# Autodesk Inventor assembly: bladesupport
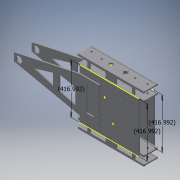
[picture p0: Inventor's stored thumbnail of the model, 180x180]
Saved by Autodesk Inventor 2017 (Build 210142000, 142)
## iProperties
Created: 2016-10-18
Part Number: bladesupport
Document SubType Name: Assembly
Designer: aesen
Author: aesen
## Documents named in this file (6)
- C:\Users\aesen\Design\for assambly\bladesupport.iam
- C:\Users\aesen\Design\for assambly\DriveTrainTop.ipt
- C:\Users\aesen\Design\for assambly\Drivetrainside.ipt
- C:\Users\aesen\Design\for assambly\DriveTrainTop_MIR.ipt
- C:\Users\aesen\Design\BattleBot-TopPlate5cmversion.ipt
- C:\Users\aesen\Design\for assambly\W1support.ipt
## Components (13 placed, 5 different names)
1. DriveTrainTop:2 — Rigid:1, Mate:4
2. Drivetrainside:1 — Rigid:1, Rigid:2
3. DriveTrainTop_MIR:1 — Rigid:2, Rigid:3, Mate:1
4. Drivetrainside:2 — Rigid:3
5. DriveTrainTop:3 — Mate:5
6. Drivetrainside:3
7. DriveTrainTop_MIR:2 — Mate:2
8. Drivetrainside:4
9. BattleBot-TopPlate5cmversion:1 — Mate:3
10. W1support:1
11. W1support:2
12. BattleBot-TopPlate5cmversion:2 — Mate:1, Mate:2, Mate:3
13. BattleBot-TopPlate5cmversion:3 — Mate:4, Mate:5
## Relationships (11: WeldJoint 6, Mate 5)
- Rigid:1 [WeldJoint]: DriveTrainTop:2 ↔ Drivetrainside:1
- Rigid:2 [WeldJoint]: Drivetrainside:1 ↔ DriveTrainTop_MIR:1
- Rigid:3 [WeldJoint]: DriveTrainTop_MIR:1 ↔ Drivetrainside:2
- [WeldJoint]: DriveTrainTop:3 ↔ Drivetrainside:3
- [WeldJoint]: Drivetrainside:3 ↔ DriveTrainTop_MIR:2
- [WeldJoint]: DriveTrainTop_MIR:2 ↔ Drivetrainside:4
- Mate:1: DriveTrainTop_MIR:1 ↔ BattleBot-TopPlate5cmversion:2
- Mate:2: DriveTrainTop_MIR:2 ↔ BattleBot-TopPlate5cmversion:2
- Mate:3: BattleBot-TopPlate5cmversion:1 ↔ BattleBot-TopPlate5cmversion:2
- Mate:4: DriveTrainTop:2 ↔ BattleBot-TopPlate5cmversion:3
- Mate:5: DriveTrainTop:3 ↔ BattleBot-TopPlate5cmversion:3
## Named parameters: d3_d2 = 0 mm, d4_d0 = 0 mm, d5_d1 = 0 mm
